# Autodesk Inventor assembly: tail_box_asembly
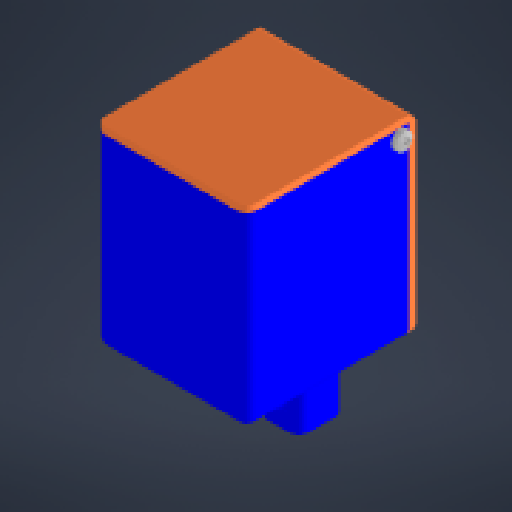
[picture p0: Inventor's stored thumbnail of the model, 512x512]
Saved by Autodesk Inventor 2024 (Build 280153000, 153)
## iProperties
Created: 2023-05-16
Part Number: tail_box_asembly
Document SubType Name: Assembly
Designer: user
Mass: 166.934 g
Surface Area: 1258.67 cm^2
Volume: 159.855 cm^3
Density: 1.04429 g/cm^3
Author: user
## Documents named in this file (5)
- D:\Docs\Robot\3d\machine_body\tail_box_asembly.iam
- D:\Docs\Robot\3d\machine_body\tail_box_asembly\tail_box.ipt
- D:\Docs\Robot\3d\electronics\bts_asembly.iam
- D:\Docs\Robot\3d\machine_body\tail_box_asembly\tail_box_cup.ipt
- C:\Users\user\Documents\Inventor\Content Center Files\R2024\ru-RU\DIN 7985 (H)\DIN 7985 (H) - M4x10-H.ipt
## Components (5 placed, 4 different names)
1. tail_box:1 — Совмещение:1, Заподлицо:1, Совмещение:2, Совмещение:3, Совмещение:4, Совмещение:5, Заподлицо:2, Заподлицо:3, Вставка:1, Вставка:2
2. bts_asembly:1 [sub-assembly] — Совмещение:3, Совмещение:4, Совмещение:5
3. tail_box_cup:1 — Заподлицо:2, Заподлицо:3
4. DIN 7985 (H) M4x10-H:1 — Вставка:1
5. DIN 7985 (H) M4x10-H:2 — Вставка:2
## Relationships (10: Mate 5, Flush 3, Insert 2)
- Совмещение:1 [Mate]: tail_box:1
- Заподлицо:1 [Flush]: tail_box:1
- Совмещение:2 [Mate]: tail_box:1
- Совмещение:3 [Mate]: tail_box:1 ↔ bts_asembly:1
- Совмещение:4 [Mate] (5 mm): tail_box:1 ↔ bts_asembly:1
- Совмещение:5 [Mate] (10 mm): tail_box:1 ↔ bts_asembly:1
- Заподлицо:2 [Flush]: tail_box:1 ↔ tail_box_cup:1
- Заподлицо:3 [Flush]: tail_box:1 ↔ tail_box_cup:1
- Вставка:1 [Insert]: tail_box:1 ↔ DIN 7985 (H) M4x10-H:1
- Вставка:2 [Insert]: tail_box:1 ↔ DIN 7985 (H) M4x10-H:2
